# Autodesk Inventor assembly: assembly
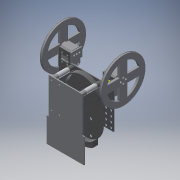
[picture p0: Inventor's stored thumbnail of the model, 180x180]
Saved by Autodesk Inventor 2016 SP1 (Build 200210100, 210)
## iProperties
Created: 2016-02-22
Part Number: assembly
Document SubType Name: Assembly
Designer: mkepler
Author: mkepler
## Documents named in this file (7)
- C:\Users\Wes\Documents\School Stuff\ECE 499\ece-499-hw1\design\mechanical\assembly.iam
- C:\Users\Wes\Documents\School Stuff\ECE 499\ece-499-hw1\design\mechanical\BaseChassis.ipt
- C:\Users\Wes\Documents\School Stuff\ECE 499\ece-499-hw1\design\mechanical\Peg.ipt
- C:\Users\Wes\Documents\School Stuff\ECE 499\ece-499-hw1\design\mechanical\TopChassis.ipt
- C:\Users\Wes\Documents\School Stuff\ECE 499\ece-499-hw1\design\mechanical\xl320Servo.ipt
- C:\Users\Wes\Documents\School Stuff\ECE 499\ece-499-hw1\design\mechanical\brace.ipt
- C:\Users\Wes\Documents\School Stuff\ECE 499\ece-499-hw1\design\mechanical\wheel.ipt
## Components (10 placed, 6 different names)
1. BaseChassis:1 — Insert:3, Mate:1, Mate:2, Insert:4, Mate:3, Insert:7, Insert:8
2. Peg:1 — Insert:3, Insert:6
3. Peg:2 — Mate:2, Mate:3, Insert:5
4. Peg:3 — Mate:1, Insert:4
5. TopChassis:1 — Insert:5, Insert:6
6. xl320Servo:1 — Insert:9, Mate:4, Insert:12, Insert:14
7. brace:1 — Insert:7, Insert:8, Insert:9, Mate:4, Insert:10, Insert:11
8. xl320Servo:2 — Insert:10, Insert:11, Insert:13, Insert:15
9. wheel:1 — Insert:12, Insert:14
10. wheel:2 — Insert:13, Insert:15
## Relationships (17: Insert 13, Mate 4)
- Insert:3: BaseChassis:1 ↔ Peg:1
- Mate:1: BaseChassis:1 ↔ Peg:3
- Mate:2: BaseChassis:1 ↔ Peg:2
- Insert:4: BaseChassis:1 ↔ Peg:3
- Mate:3: BaseChassis:1 ↔ Peg:2
- Insert:5: Peg:2 ↔ TopChassis:1
- Insert:6: Peg:1 ↔ TopChassis:1
- Insert:7: BaseChassis:1 ↔ brace:1
- Insert:8: BaseChassis:1 ↔ brace:1
- Insert:9: xl320Servo:1 ↔ brace:1
- Mate:4: xl320Servo:1 ↔ brace:1
- Insert:10: brace:1 ↔ xl320Servo:2
- Insert:11: brace:1 ↔ xl320Servo:2
- Insert:12: xl320Servo:1 ↔ wheel:1
- Insert:13: xl320Servo:2 ↔ wheel:2
- Insert:14: xl320Servo:1 ↔ wheel:1
- Insert:15: xl320Servo:2 ↔ wheel:2
